# Autodesk Inventor assembly: 1A.01.01.02-HB-Wing Assembly2
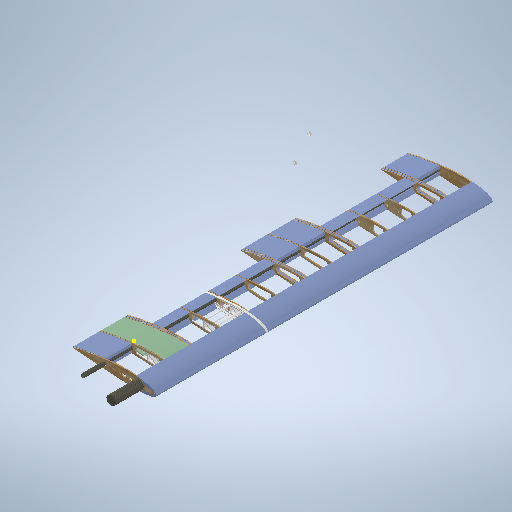
[picture p0: Inventor's stored thumbnail of the model, 512x512]
Saved by Autodesk Inventor 2025.2 (Build 292293000, 293)
## iProperties
Created: 2024-12-29
Part Number: 1A.01.01.02-HB-Wing Assembly2
Document SubType Name: Assembly
Designer: hjbre
Author: hjbre
## Documents named in this file (36)
- C:\Users\Imist\OneDrive - University of Bristol\Year 2\AVDASI 2\Team\Final CAD\1A.01.01.02-HB-Wing Assembly2.iam
- C:\Users\Imist\OneDrive - University of Bristol\Year 2\AVDASI 2\Team\Final CAD\1P.01.01.01-HB-Rib1.ipt
- C:\Users\Imist\OneDrive - University of Bristol\Year 2\AVDASI 2\Team\Final CAD\1P.01.01.02-HB-Rib2.ipt
- C:\Users\Imist\OneDrive - University of Bristol\Year 2\AVDASI 2\Team\Final CAD\1P.01.01.03-HB-Rib3.ipt
- C:\Users\Imist\OneDrive - University of Bristol\Year 2\AVDASI 2\Team\Final CAD\1P.01.01.04-HB-Rib4.ipt
- C:\Users\Imist\OneDrive - University of Bristol\Year 2\AVDASI 2\Team\Final CAD\1P.01.01.05-HB-Rib5.ipt
- C:\Users\Imist\OneDrive - University of Bristol\Year 2\AVDASI 2\Team\Final CAD\1P.02.01.01-HB-FalseRearSpar.ipt
- C:\Users\Imist\OneDrive - University of Bristol\Year 2\AVDASI 2\Team\Final CAD\1P.01.01.06-HB-Rib6.ipt
- C:\Users\Imist\OneDrive - University of Bristol\Year 2\AVDASI 2\Team\Final CAD\1P.01.01.07-HB-Rib7.ipt
- C:\Users\Imist\OneDrive - University of Bristol\Year 2\AVDASI 2\Team\Final CAD\1P.01.01.08-HB-Rib8.ipt
- C:\Users\Imist\OneDrive - University of Bristol\Year 2\AVDASI 2\Team\Final CAD\1P.01.01.09-HB-Rib9.ipt
- C:\Users\Imist\OneDrive - University of Bristol\Year 2\AVDASI 2\Team\Final CAD\1P.01.01.10-HB-Rib10a.ipt
- C:\Users\Imist\OneDrive - University of Bristol\Year 2\AVDASI 2\Team\Final CAD\1P.01.01.11-HB-Rib11.ipt
- C:\Users\Imist\OneDrive - University of Bristol\Year 2\AVDASI 2\Team\Final CAD\1P.01.01.12-HB-Rib12.ipt
- C:\Users\Imist\OneDrive - University of Bristol\Year 2\AVDASI 2\Team\Final CAD\1P.01.01.13-HB-Rib13.ipt
- C:\Users\Imist\OneDrive - University of Bristol\Year 2\AVDASI 2\Team\Final CAD\Skin.ipt
- C:\Users\Imist\OneDrive - University of Bristol\Year 2\AVDASI 2\Team\Final CAD\1P.01.02.01-HB-TrailingEdgeRootEnd.ipt
- C:\Users\Imist\OneDrive - University of Bristol\Year 2\AVDASI 2\Team\Final CAD\1P.01.02.02-HB-TrailingEdgeSand-Rib.ipt
- C:\Users\Imist\OneDrive - University of Bristol\Year 2\AVDASI 2\Team\Final CAD\1P.01.04.01-HB-Rib3Foam.ipt
- C:\Users\Imist\OneDrive - University of Bristol\Year 2\AVDASI 2\Team\Final CAD\1P.01.04.02-HB-Rib7Foam.ipt
- C:\Users\Imist\OneDrive - University of Bristol\Year 2\AVDASI 2\Team\Final CAD\1P.01.04.03-HB-Rib9Foam.ipt
- C:\Users\Imist\OneDrive - University of Bristol\Year 2\AVDASI 2\Team\Final CAD\1P.01.04.04-HB-Rib12Foam.ipt
- C:\Users\Imist\OneDrive - University of Bristol\Year 2\AVDASI 2\Team\Final CAD\1P.01.02.03-HB-TrailingEdgeTipEnd.ipt
- C:\Users\Imist\OneDrive - University of Bristol\Year 2\AVDASI 2\Team\Final CAD\1P.01.03.04-HB-AileronFoamOuter.ipt
- C:\Users\Imist\OneDrive - University of Bristol\Year 2\AVDASI 2\Team\Final CAD\1P.01.03.05-HB-AileronFoamInner.ipt
- C:\Users\Imist\OneDrive - University of Bristol\Year 2\AVDASI 2\Team\Final CAD\1P.01.03.01-HB-FlapFoamOuter.ipt
- C:\Users\Imist\OneDrive - University of Bristol\Year 2\AVDASI 2\Team\Final CAD\1P.01.03.03-HB-FlapFoam.ipt
- C:\Users\Imist\OneDrive - University of Bristol\Year 2\AVDASI 2\Team\Final CAD\1P.01.05.01-HB-PressureTap.ipt
- C:\Users\Imist\OneDrive - University of Bristol\Year 2\AVDASI 2\Team\Final CAD\1P.01.03.02-HB-FlapFoamPressTap.ipt
- C:\Users\Imist\OneDrive - University of Bristol\Year 2\AVDASI 2\Team\Final CAD\1P.01.02.05-HB-LeadingEdgeTipEnd.ipt
- C:\Users\Imist\OneDrive - University of Bristol\Year 2\AVDASI 2\Team\Final CAD\1P.01.02.04-HB-LeadingEdgeRootEnd.ipt
- C:\Users\Imist\OneDrive - University of Bristol\Year 2\AVDASI 2\Team\Final CAD\1P.02.01.02-RN-MainSpar.ipt
- C:\Users\Imist\OneDrive - University of Bristol\Year 2\AVDASI 2\Team\Final CAD\1P.01.05.03-HB-PlatformFinal.ipt
- C:\Users\Imist\OneDrive - University of Bristol\Year 2\AVDASI 2\Team\Final CAD\1P.01.02.06-HB-Trailing adge access panel.ipt
- C:\Users\Imist\OneDrive - University of Bristol\Year 2\AVDASI 2\Team\Final CAD\1P.01.05.04-HB-PlatformFinala.ipt
- C:\Users\Imist\OneDrive - University of Bristol\Year 2\AVDASI 2\Team\Final CAD\2P.03.01.00.05.IM.Bearing8123.5.ipt
## Components (45 placed, 35 different names)
1. Skin:1 — Insert:21
2. 1P.02.01.02-RN-MainSpar:1 — Insert:47
3. 1P.01.05.03-HB-PlatformFinal:1 — Insert:48
4. 1P.01.02.06-HB-Trailing adge access panel:1 — Insert:49
5. 1P.01.05.04-HB-PlatformFinala:1 — Insert:50
6. 2P.03.01.00.05.IM.Bearing8123.5:1
7. 2P.03.01.00.05.IM.Bearing8123.5:2
8. 2P.03.01.00.05.IM.Bearing8123.5:3
9. 2P.03.01.00.05.IM.Bearing8123.5:4
10. 1P.02.01.01-HB-FalseRearSpar:1 — Insert:9
11. 1P.01.02.04-HB-LeadingEdgeRootEnd:1 — Insert:46
12. 1P.01.02.05-HB-LeadingEdgeTipEnd:1 — Insert:45
13. 1P.01.03.02-HB-FlapFoamPressTap:1 — Insert:42
14. 1P.01.03.01-HB-FlapFoamOuter:2 — Insert:39
15. 1P.01.03.03-HB-FlapFoam:1 — Mate:2
16. 1P.01.03.01-HB-FlapFoamOuter:1 — Insert:38
17. 1P.01.03.05-HB-AileronFoamInner:1 — Insert:36
18. 1P.01.03.04-HB-AileronFoamOuter:2 — Insert:35
19. 1P.01.03.04-HB-AileronFoamOuter:1 — Insert:37
20. 1P.01.02.01-HB-TrailingEdgeRootEnd:1 — Insert:22
21. 1P.01.02.02-HB-TrailingEdgeSand-Rib:2 — Insert:28
22. 1P.01.02.02-HB-TrailingEdgeSand-Rib:3 — Insert:29
23. 1P.01.02.03-HB-TrailingEdgeTipEnd:1 — Insert:33
24. 1P.01.05.01-HB-PressureTap:1 — Insert:41, Insert:42
25. 1P.01.01.11-HB-Rib11:1 — Insert:34, Insert:37, Insert:43
26. 1P.01.01.01-HB-Rib1:1 — Insert:1, Insert:9, Insert:21, Insert:22, Insert:46
27. 1P.01.01.02-HB-Rib2:1 — Insert:1, Insert:2, Insert:48
28. 1P.01.01.03-HB-Rib3:1 — Insert:2, Insert:24, Insert:49
29. 1P.01.01.04-HB-Rib4:1 — Insert:3, Insert:4, Insert:50
30. 1P.01.01.05-HB-Rib5:1 — Insert:4, Insert:10, Mate:2, Insert:41, Insert:45
31. 1P.01.01.06-HB-Rib6:1 — Insert:10, Insert:11, Insert:38
32. 1P.01.01.07-HB-Rib7:1 — Insert:11, Insert:26
33. 1P.01.01.08-HB-Rib8:1 — Insert:12, Insert:13, Insert:29
34. 1P.01.01.09-HB-Rib9:1 — Insert:13, Insert:30
35. 1P.01.01.10-HB-Rib10a:1 — Insert:16, Insert:34, Insert:36
36. 1P.01.01.12-HB-Rib12:1 — Mate:1, Insert:43
37. 1P.01.01.13-HB-Rib13:1 — Insert:19, Insert:47
38. 1P.01.04.01-HB-Rib3Foam:1 — Insert:24, Insert:25
39. 1P.01.01.03-HB-Rib3:2 — Insert:25, Insert:3, Insert:39
40. 1P.01.04.02-HB-Rib7Foam:1 — Insert:26, Insert:27
41. 1P.01.01.07-HB-Rib7:2 — Insert:27, Insert:28, Insert:12
42. 1P.01.04.03-HB-Rib9Foam:1 — Insert:30, Insert:31
43. 1P.01.01.09-HB-Rib9:2 — Insert:31, Insert:16, Insert:35
44. 1P.01.04.04-HB-Rib12Foam:1 — Mate:1, Insert:32
45. 1P.01.01.12-HB-Rib12:2 — Insert:32, Insert:19, Insert:33
## Relationships (40: Insert 38, Mate 2)
- Insert:1 (94 mm): 1P.01.01.01-HB-Rib1:1 ↔ 1P.01.01.02-HB-Rib2:1
- Insert:2 (85 mm): 1P.01.01.02-HB-Rib2:1 ↔ 1P.01.01.03-HB-Rib3:1
- Insert:3 (98 mm): 1P.01.01.04-HB-Rib4:1 ↔ 1P.01.01.03-HB-Rib3:2
- Insert:4 (96 mm): 1P.01.01.04-HB-Rib4:1 ↔ 1P.01.01.05-HB-Rib5:1
- Insert:9: 1P.02.01.01-HB-FalseRearSpar:1 ↔ 1P.01.01.01-HB-Rib1:1
- Insert:10 (96 mm): 1P.01.01.05-HB-Rib5:1 ↔ 1P.01.01.06-HB-Rib6:1
- Insert:11 (98 mm): 1P.01.01.06-HB-Rib6:1 ↔ 1P.01.01.07-HB-Rib7:1
- Insert:12 (85 mm): 1P.01.01.08-HB-Rib8:1 ↔ 1P.01.01.07-HB-Rib7:2
- Insert:13 (85 mm): 1P.01.01.08-HB-Rib8:1 ↔ 1P.01.01.09-HB-Rib9:1
- Insert:16 (98 mm): 1P.01.01.10-HB-Rib10a:1 ↔ 1P.01.01.09-HB-Rib9:2
- Insert:19 (83 mm): 1P.01.01.13-HB-Rib13:1 ↔ 1P.01.01.12-HB-Rib12:2
- Insert:21: Skin:1 ↔ 1P.01.01.01-HB-Rib1:1
- Insert:22: 1P.01.02.01-HB-TrailingEdgeRootEnd:1 ↔ 1P.01.01.01-HB-Rib1:1
- Insert:24: 1P.01.01.03-HB-Rib3:1 ↔ 1P.01.04.01-HB-Rib3Foam:1
- Insert:25: 1P.01.04.01-HB-Rib3Foam:1 ↔ 1P.01.01.03-HB-Rib3:2
- Insert:26: 1P.01.01.07-HB-Rib7:1 ↔ 1P.01.04.02-HB-Rib7Foam:1
- Insert:27: 1P.01.04.02-HB-Rib7Foam:1 ↔ 1P.01.01.07-HB-Rib7:2
- Insert:28: 1P.01.02.02-HB-TrailingEdgeSand-Rib:2 ↔ 1P.01.01.07-HB-Rib7:2
- Insert:29: 1P.01.02.02-HB-TrailingEdgeSand-Rib:3 ↔ 1P.01.01.08-HB-Rib8:1
- Insert:30: 1P.01.01.09-HB-Rib9:1 ↔ 1P.01.04.03-HB-Rib9Foam:1
- Insert:31: 1P.01.04.03-HB-Rib9Foam:1 ↔ 1P.01.01.09-HB-Rib9:2
- Mate:1: 1P.01.01.12-HB-Rib12:1 ↔ 1P.01.04.04-HB-Rib12Foam:1
- Insert:32: 1P.01.04.04-HB-Rib12Foam:1 ↔ 1P.01.01.12-HB-Rib12:2
- Insert:33: 1P.01.02.03-HB-TrailingEdgeTipEnd:1 ↔ 1P.01.01.12-HB-Rib12:2
- Insert:34 (96 mm): 1P.01.01.11-HB-Rib11:1 ↔ 1P.01.01.10-HB-Rib10a:1
- Insert:35: 1P.01.03.04-HB-AileronFoamOuter:2 ↔ 1P.01.01.09-HB-Rib9:2
- Insert:36: 1P.01.03.05-HB-AileronFoamInner:1 ↔ 1P.01.01.10-HB-Rib10a:1
- Insert:37: 1P.01.03.04-HB-AileronFoamOuter:1 ↔ 1P.01.01.11-HB-Rib11:1
- Insert:38: 1P.01.03.01-HB-FlapFoamOuter:1 ↔ 1P.01.01.06-HB-Rib6:1
- Insert:39: 1P.01.03.01-HB-FlapFoamOuter:2 ↔ 1P.01.01.03-HB-Rib3:2
- Mate:2: 1P.01.03.03-HB-FlapFoam:1 ↔ 1P.01.01.05-HB-Rib5:1
- Insert:41: 1P.01.05.01-HB-PressureTap:1 ↔ 1P.01.01.05-HB-Rib5:1
- Insert:42: 1P.01.03.02-HB-FlapFoamPressTap:1 ↔ 1P.01.05.01-HB-PressureTap:1
- Insert:43 (98 mm): 1P.01.01.11-HB-Rib11:1 ↔ 1P.01.01.12-HB-Rib12:1
- Insert:45: 1P.01.02.05-HB-LeadingEdgeTipEnd:1 ↔ 1P.01.01.05-HB-Rib5:1
- Insert:46: 1P.01.02.04-HB-LeadingEdgeRootEnd:1 ↔ 1P.01.01.01-HB-Rib1:1
- Insert:47: 1P.02.01.02-RN-MainSpar:1 ↔ 1P.01.01.13-HB-Rib13:1
- Insert:48: 1P.01.05.03-HB-PlatformFinal:1 ↔ 1P.01.01.02-HB-Rib2:1
- Insert:49: 1P.01.02.06-HB-Trailing adge access panel:1 ↔ 1P.01.01.03-HB-Rib3:1
- Insert:50: 1P.01.05.04-HB-PlatformFinala:1 ↔ 1P.01.01.04-HB-Rib4:1
## Named parameters: Finish10_Area = 15008.3, Finish10_Thickness = 0.05 mm, Finish11_Area = 15008.3, Finish11_Thickness = 0.05 mm, Finish12_Area = 15008.3, Finish12_Thickness = 0.05 mm, Finish13_Area = 15008.3, Finish14_Area = 15008.3, Finish15_Area = 1601.78, Finish16_Area = 147.262, Finish16_Thickness = 0.05 mm, Finish17_Area = 564.44, Finish17_Thickness = 0.05 mm, Finish18_Area = 274.875, Finish19_Area = 904.49, Finish19_Thickness = 0.05 mm, Finish1_Area = 646.44, Finish1_Thickness = 0.05 mm, Finish20_Area = 138.949, Finish21_Area = 150.143, Finish21_Thickness = 0.05 mm, Finish22_Area = 139.779, Finish23_Area = 369.074, Finish23_Thickness = 0.05 mm, Finish24_Area = 124.798, Finish25_Area = 548.598, Finish25_Thickness = 0.05 mm, Finish26_Area = 475.518, Finish26_Thickness = 0.05 mm, Finish27_Area = 4059.13, Finish27_Thickness = 0.05 mm, Finish28_Area = 1152.31, Finish29_Area = 843.033, Finish29_Thickness = 0.05 mm, Finish7_Area = 728.581
note: some values were not read from the file. Shown as the stored number, unit unknown: "Finish10_Area", "Finish11_Area", "Finish12_Area", "Finish13_Area", "Finish14_Area", "Finish15_Area", "Finish16_Area", "Finish17_Area", "Finish18_Area", "Finish19_Area", "Finish1_Area", "Finish20_Area", "Finish21_Area", "Finish22_Area", "Finish23_Area", "Finish24_Area", "Finish25_Area", "Finish26_Area", "Finish27_Area", "Finish28_Area", "Finish29_Area", "Finish7_Area".
